# Autodesk Inventor assembly: BuildAssem
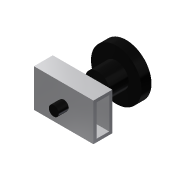
[picture p0: Inventor's stored thumbnail of the model, 180x180]
Saved by Autodesk Inventor 2014 (Build 180170000, 170)
## iProperties
Created: 2014-08-10
Part Number: BuildAssem
Document SubType Name: Assembly
Designer: Peele
Author: Peele
## Documents named in this file (3)
- E:\Copy\DLP\Concept\SubAssem\BuildAssem.iam
- E:\Copy\DLP\Concept\StockParts\AluminumBlock.ipt
- E:\Copy\DLP\Concept\StockParts\Knob.ipt
## Components (2 placed, 2 different names)
1. AluminumBlock:1 — Mate:1, Mate:2
2. Knob:1 — Mate:1, Mate:2
## Relationships (2: Mate 2)
- Mate:1 (15 mm): AluminumBlock:1 ↔ Knob:1
- Mate:2: AluminumBlock:1 ↔ Knob:1
